# Autodesk Inventor assembly: Lift Assembly
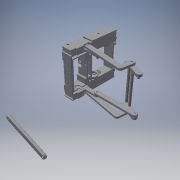
[picture p0: Inventor's stored thumbnail of the model, 180x180]
Saved by Autodesk Inventor 2017 (Build 210142000, 142)
## iProperties
Created: 2017-08-13
Part Number: Lift Assembly
Document SubType Name: Assembly
Designer: Dale
Author: Dale
## Documents named in this file (7)
- C:\Users\Dale\saved\Projects\Scrambler\Assemblies\Lift Assembly.iam
- C:\Users\Dale\saved\Projects\Scrambler\3D_Printed\CAD\Body\Chassis.ipt
- C:\Users\Dale\saved\Projects\Scrambler\3D_Printed\CAD\Manipulator\Lift Mount Right.ipt
- C:\Users\Dale\saved\Projects\Scrambler\3D_Printed\CAD\Manipulator\Lift Mount Right_MIR.ipt
- C:\Users\Dale\saved\Projects\Scrambler\3D_Printed\CAD\Manipulator\Lift Arm Lower.ipt
- C:\Users\Dale\saved\Projects\Scrambler\3D_Printed\CAD\Manipulator\Front Push Bar.ipt
- C:\Users\Dale\saved\Projects\Scrambler\3D_Printed\CAD\Manipulator\Lift Arm Upper2.ipt
## Components (8 placed, 6 different names)
1. Chassis:1 — Mate:1, Mate:2, Mate:3, Mate:4, Mate:5, Mate:6
2. Lift Mount Right:1 — Mate:1, Mate:2, Mate:3, Rotational:3, Rotational:5
3. Lift Mount Right_MIR:1 — Mate:4, Mate:5, Mate:6, Rotational:2
4. Lift Arm Lower:1 — Rotational:3, Rotational:4
5. Lift Arm Lower:2 — Rotational:2, Cylindrical:1
6. Front Push Bar:1 — Rotational:4, Cylindrical:1, Rotational:6
7. Lift Arm Upper2:1
8. Lift Arm Upper2:2 — Rotational:5, Rotational:6
## Relationships (12: Mate 6, RevoluteJoint 5, CylindricalJoint 1)
- Mate:1: Chassis:1 ↔ Lift Mount Right:1
- Mate:2: Chassis:1 ↔ Lift Mount Right:1
- Mate:3: Chassis:1 ↔ Lift Mount Right:1
- Mate:4: Chassis:1 ↔ Lift Mount Right_MIR:1
- Mate:5: Chassis:1 ↔ Lift Mount Right_MIR:1
- Mate:6: Chassis:1 ↔ Lift Mount Right_MIR:1
- Rotational:2 [RevoluteJoint]: Lift Mount Right_MIR:1 ↔ Lift Arm Lower:2
- Rotational:3 [RevoluteJoint]: Lift Mount Right:1 ↔ Lift Arm Lower:1
- Rotational:4 [RevoluteJoint] (-2 mm): Lift Arm Lower:1 ↔ Front Push Bar:1
- Cylindrical:1: Lift Arm Lower:2 ↔ Front Push Bar:1
- Rotational:5 [RevoluteJoint]: Lift Mount Right:1 ↔ Lift Arm Upper2:2
- Rotational:6 [RevoluteJoint]: Front Push Bar:1 ↔ Lift Arm Upper2:2
